# Autodesk Inventor assembly: Sessao_08_04
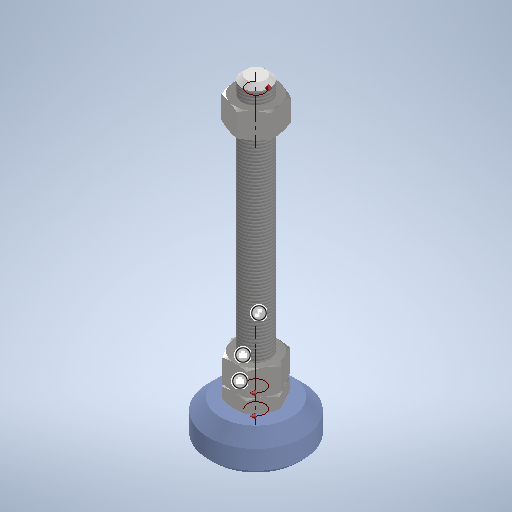
[picture p0: Inventor's stored thumbnail of the model, 512x512]
Saved by Autodesk Inventor 2026 (Build 300175000, 175)
## iProperties
Created: 2025-04-08
Part Number: Sessao_08_04
Document SubType Name: Assembly
Designer: Carlos Dias
Author: Carlos Dias
## Documents named in this file (5)
- C:\Users\Carlos Dias\Documents\Formação-TEARCI\UFCDs\5134 - Robótica _ Fundamentos\Material De Apoio\Sessao_08_04\Sessao_08_04_999_001.iam
- C:\Users\Carlos Dias\Documents\Formação-TEARCI\UFCDs\5134 - Robótica _ Fundamentos\Material De Apoio\Sessao_08_04\peça_001_001.ipt
- C:\Users\Carlos Dias\Documents\Formação-TEARCI\UFCDs\5134 - Robótica _ Fundamentos\Material De Apoio\Sessao_08_04\peça_002_001.ipt
- C:\Users\Carlos Dias\Documents\Inventor\Content Center Files\R2026\en-US\ANSI B18.2.4.5M\ANSI B18.2.4.5M - M12 x 1.75.ipt
- C:\Users\Carlos Dias\Documents\Inventor\Content Center Files\R2026\en-US\ANSI B 18.2.4.1 M(1)\ANSI B 18.2.4.1 M - M12 x 1,75Style 1.ipt
## Components (5 placed, 4 different names)
1. peça_001_001:1 — Flush:1, Flush:2, Flush:3, Mate:1, Mate:2, Mate:4
2. peça_002_001:1 — Mate:1, Mate:2, Mate:3, Mate:5, Mate:7, Flush:4, Flush:5
3. Hex Jam Nut - Metric M12 x 1.75:1 — Mate:3, Mate:4, Mate:6
4. Hex Nut Metric M12 x 1,75:1 — Mate:5, Mate:6
5. Hex Nut Metric M12 x 1,75:2 — Mate:7, Flush:4
## Relationships (12: Mate 7, Flush 5)
- Flush:1: peça_001_001:1
- Flush:2: peça_001_001:1
- Flush:3: peça_001_001:1
- Mate:1: peça_001_001:1 ↔ peça_002_001:1
- Mate:2: peça_001_001:1 ↔ peça_002_001:1
- Mate:3: peça_002_001:1 ↔ Hex Jam Nut - Metric M12 x 1.75:1
- Mate:4: peça_001_001:1 ↔ Hex Jam Nut - Metric M12 x 1.75:1
- Mate:5: peça_002_001:1 ↔ Hex Nut Metric M12 x 1,75:1
- Mate:6: Hex Jam Nut - Metric M12 x 1.75:1 ↔ Hex Nut Metric M12 x 1,75:1
- Mate:7: peça_002_001:1 ↔ Hex Nut Metric M12 x 1,75:2
- Flush:4 (7.089 mm): peça_002_001:1 ↔ Hex Nut Metric M12 x 1,75:2
- Flush:5: peça_002_001:1
